# Autodesk Inventor assembly: Leg V3
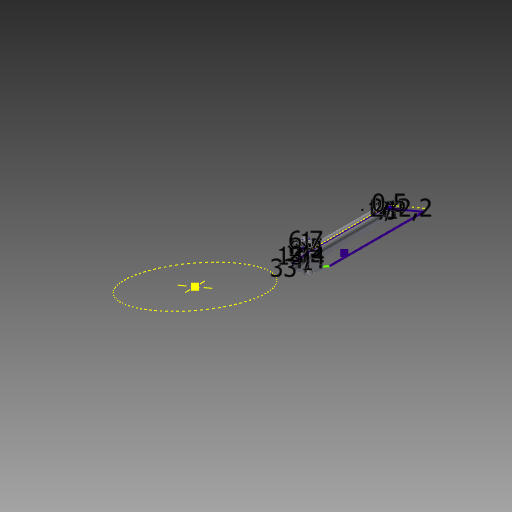
[picture p0: Inventor's stored thumbnail of the model, 512x512]
Saved by Autodesk Inventor 2019.1 (Build 231200000, 200)
## iProperties
Created: 2018-11-20
Part Number: Leg V3
Material: Generisch
Document SubType Name: Assembly
Designer: JochenAlt
Author: JochenAlt
## Documents named in this file (5)
- D:\Projects\Ondine\CAD\Leg\Leg V3.iam
- D:\Projects\Ondine\CAD\Leg\Leg V3.ipt
- D:\Projects\Ondine\CAD\Leg\Schnecke\Schneckenrad1.ipt
- D:\Projects\Ondine\CAD\Bearings\W 637_4 X.iam
- D:\Projects\Ondine\CAD\Leg\LegInnerGear\LegV3Axis1.ipt
## Components (5 placed, 4 different names)
1. Leg:1 — Passend:5, Winkel:1, Passend:6, Passend:11
2. LegGearWormPinion:1 — Passend:5, Winkel:1, Passend:6, Passend:7, Passend:10
3. LegV3Axis1:1 — Passend:7, Passend:8, Passend:9
4. W 637_4 X:1 [sub-assembly] — Passend:8, Passend:11
5. W 637_4 X:2 [sub-assembly] — Passend:9, Passend:10
## Relationships (8: Mate 7, Angle 1)
- Passend:5 [Mate]: Leg:1 ↔ LegGearWormPinion:1
- Winkel:1 [Angle] (0 deg): Leg:1 ↔ LegGearWormPinion:1
- Passend:6 [Mate]: Leg:1 ↔ LegGearWormPinion:1
- Passend:7 [Mate]: LegGearWormPinion:1 ↔ LegV3Axis1:1
- Passend:8 [Mate]: LegV3Axis1:1 ↔ W 637_4 X:1
- Passend:9 [Mate]: LegV3Axis1:1 ↔ W 637_4 X:2
- Passend:10 [Mate]: LegGearWormPinion:1 ↔ W 637_4 X:2
- Passend:11 [Mate]: Leg:1 ↔ W 637_4 X:1
